# Autodesk Inventor assembly: back_platform_assembly_without_window
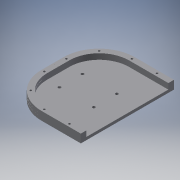
[picture p0: Inventor's stored thumbnail of the model, 180x180]
Saved by Autodesk Inventor 2016 (Build 200138000, 138)
## iProperties
Created: 2015-09-09
Part Number: back_platform_assembly_without_window
Document SubType Name: Assembly
Designer: oscar
Author: oscar
## Documents named in this file (3)
- C:\Users\oscar\Desktop\technical_drawings\youbot\back_platform\v1.0\inventor_parts\back_platform_assembly_without_window.iam
- C:\Users\oscar\Desktop\technical_drawings\youbot\back_platform\v1.0\inventor_parts\back_platform_without_window.ipt
- C:\Users\oscar\Desktop\technical_drawings\youbot\back_platform\v1.0\inventor_parts\side_walls.ipt
## Components (5 placed, 2 different names)
1. back_platform_without_window:1 — Mate:1, Flush:1, Flush:4, Mate:5, Flush:7, Flush:8, Mate:6, Flush:9, Mate:7
2. side_walls:1 — Mate:2, Flush:2, Flush:3
3. side_walls:2 — Mate:1, Mate:2, Flush:1, Flush:2, Flush:3, Flush:4
4. side_walls:3 — Mate:4, Flush:5, Flush:6, Flush:7
5. side_walls:4 — Mate:4, Mate:5, Flush:5, Flush:6, Flush:8
## Relationships (15: Flush 9, Mate 6)
- Mate:1: back_platform_without_window:1 ↔ side_walls:2
- Mate:2: side_walls:1 ↔ side_walls:2
- Mate:4: side_walls:3 ↔ side_walls:4
- Flush:1: back_platform_without_window:1 ↔ side_walls:2
- Flush:2: side_walls:1 ↔ side_walls:2
- Flush:3: side_walls:1 ↔ side_walls:2
- Flush:4: back_platform_without_window:1 ↔ side_walls:2
- Mate:5: back_platform_without_window:1 ↔ side_walls:4
- Flush:5: side_walls:3 ↔ side_walls:4
- Flush:6: side_walls:3 ↔ side_walls:4
- Flush:7: back_platform_without_window:1 ↔ side_walls:3
- Flush:8: back_platform_without_window:1 ↔ side_walls:4
- Mate:6: back_platform_without_window:1
- Flush:9: back_platform_without_window:1
- Mate:7: back_platform_without_window:1
